# Autodesk Inventor assembly: CombinedSensorMount
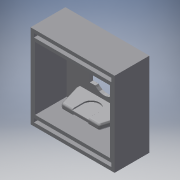
[picture p0: Inventor's stored thumbnail of the model, 180x180]
Saved by Autodesk Inventor 2017 (Build 210142000, 142)
## iProperties
Created: 2017-02-05
Part Number: CombinedSensorMount
Document SubType Name: Assembly
Designer: Moonlight.Admin
Author: Moonlight.Admin
## Documents named in this file (3)
- D:\Documents\DIY Projects\FRC3941\CombinedSensorMount.iam
- C:\Users\Moonlight.Admin\Documents\lifecammountplain.ipt
- C:\Users\Moonlight.Admin\Documents\Housing.ipt
## Components (2 placed, 2 different names)
1. lifecammountplain:1 — Mate:1
2. Housing:1 — Flush:1
## Relationships (2: Mate 1, Flush 1)
- Mate:1: lifecammountplain:1
- Flush:1: Housing:1
